# Autodesk Inventor assembly: periscope
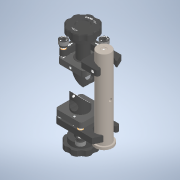
[picture p0: Inventor's stored thumbnail of the model, 180x180]
Saved by Autodesk Inventor 2021 (Build 250183000, 183)
## iProperties
Created: 2020-06-18
Part Number: periscope
Document SubType Name: Assembly
Designer: Saumya
Author: Saumya
## Documents named in this file (5)
- C:\Users\Saumya\Documents\Inventor\ClearedTissue\clear tissue_2_cad\Components\Assemblies\periscope.iam
- C:\Users\Saumya\Documents\Inventor\ClearedTissue\clear tissue_2_cad\Components\ThorLabs\RS6P8E.ipt
- C:\Users\Saumya\Documents\Inventor\ClearedTissue\clear tissue_2_cad\Components\ThorLabs\RS99T.ipt
- C:\Users\Saumya\Documents\Inventor\ClearedTissue\clear tissue_2_cad\Components\ThorLabs\H45B2.ipt
- C:\Users\Saumya\Documents\Inventor\ClearedTissue\clear tissue_2_cad\Components\ThorLabs\PF10-03-P01.ipt
## Components (7 placed, 4 different names)
1. RS6P8E:1
2. RS99T:2 — Mate:2
3. RS99T:3 — Mate:1
4. H45B2:1 — Mate:1, Rotational:2
5. H45B2:2 — Mate:2, Rotational:1
6. PF10-03-P01:1 — Rotational:2
7. PF10-03-P01:2 — Rotational:1
## Relationships (4: Mate 2, RevoluteJoint 2)
- Mate:1: RS99T:3 ↔ H45B2:1
- Mate:2: RS99T:2 ↔ H45B2:2
- Rotational:1 [RevoluteJoint]: H45B2:2 ↔ PF10-03-P01:2
- Rotational:2 [RevoluteJoint]: H45B2:1 ↔ PF10-03-P01:1
